# Autodesk Inventor assembly: Soporte_chumacera
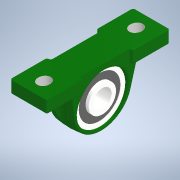
[picture p0: Inventor's stored thumbnail of the model, 180x180]
Saved by Autodesk Inventor 2020 (Build 240168000, 168)
## iProperties
Created: 2021-01-14
Part Number: Soporte_chumacera
Document SubType Name: Assembly
Designer: Cerberus 1S
Author: Cerberus 1S
## Documents named in this file (3)
- C:\Users\Cerberus 1S\Universidad de los Andes\Robocol - Documentos\Sub Tracción\Chasis\Diseño 1.3 (2020)\Soporte_chumacera.iam
- C:\Users\Cerberus 1S\Universidad de los Andes\Robocol - Documentos\Sub Tracción\Chasis\Diseño 1.3 (2020)\Extrusion de prueba.ipt
- C:\Users\Cerberus 1S\Universidad de los Andes\Robocol - Documentos\Sub Tracción\Chasis\Diseño 1.3 (2020)\AST_Bearings_UCP204-12_MIR1.ipt
## Components (2 placed, 2 different names)
1. Extrusion de prueba:1 — Coincidencia:1, Coincidencia:2, Nivelación:1
2. AST_Bearings_UCP204-12_MIR1:1 — Coincidencia:1, Coincidencia:2, Nivelación:1
## Relationships (3: Mate 2, Flush 1)
- Coincidencia:1 [Mate]: Extrusion de prueba:1 ↔ AST_Bearings_UCP204-12_MIR1:1
- Coincidencia:2 [Mate] (-29 mm): Extrusion de prueba:1 ↔ AST_Bearings_UCP204-12_MIR1:1
- Nivelación:1 [Flush] (80 mm): Extrusion de prueba:1 ↔ AST_Bearings_UCP204-12_MIR1:1
